# Autodesk Inventor assembly: docisk poprawne
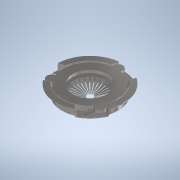
[picture p0: Inventor's stored thumbnail of the model, 180x180]
Saved by Autodesk Inventor 2022 (Build 260153000, 153)
## iProperties
Created: 2021-05-23
Part Number: docisk poprawne
Document SubType Name: Assembly
Designer: Matik
Author: Matik
## Documents named in this file (7)
- C:\Users\Mateu\Desktop\Modele\ClutchPressurePlate.iam
- C:\Users\Mateu\Desktop\Modele\ClutchPressurePlate_Casting.ipt
- C:\Users\Mateu\Desktop\Modele\ClutchPressurePlate_PlateSpring.ipt
- C:\Users\Mateu\Desktop\Modele\ClutchPressurePlate_TapeSpring.ipt
- C:\Users\Mateu\Desktop\Modele\ClutchPressurePlate_Cover.ipt
- C:\Users\Mateu\Desktop\Modele\ClutchPressurePlate_Rivet.ipt
- C:\Users\Mateu\Desktop\Modele\ClutchPressurePlate_RivetLong.ipt
## Components (12 placed, 6 different names)
1. ClutchPressurePlate_Casting:1 — Wstawiające:1, Wstawiające:2, Wstawiające:3, Wstawiające:4, Wstawiające:13
2. ClutchPressurePlate_PlateSpring:1 — Wstawiające:1
3. ClutchPressurePlate_TapeSpring:1 — Wstawiające:2, Wstawiające:6, Wstawiające:11
4. ClutchPressurePlate_TapeSpring:2 — Wstawiające:4, Wstawiające:7, Wstawiające:12
5. ClutchPressurePlate_TapeSpring:3 — Wstawiające:3, Wstawiające:5
6. ClutchPressurePlate_Cover:1 — Wstawiające:5, Wstawiające:6, Wstawiające:7, Wstawiające:8, Wstawiające:9, Wstawiające:10
7. ClutchPressurePlate_Rivet:1 — Wstawiające:8
8. ClutchPressurePlate_Rivet:2 — Wstawiające:9
9. ClutchPressurePlate_Rivet:3 — Wstawiające:10
10. ClutchPressurePlate_RivetLong:1 — Wstawiające:11
11. ClutchPressurePlate_RivetLong:2 — Wstawiające:13
12. ClutchPressurePlate_RivetLong:3 — Wstawiające:12
## Relationships (13: Insert 13)
- Wstawiające:1 [Insert]: ClutchPressurePlate_Casting:1 ↔ ClutchPressurePlate_PlateSpring:1
- Wstawiające:2 [Insert]: ClutchPressurePlate_Casting:1 ↔ ClutchPressurePlate_TapeSpring:1
- Wstawiające:3 [Insert]: ClutchPressurePlate_Casting:1 ↔ ClutchPressurePlate_TapeSpring:3
- Wstawiające:4 [Insert]: ClutchPressurePlate_Casting:1 ↔ ClutchPressurePlate_TapeSpring:2
- Wstawiające:5 [Insert]: ClutchPressurePlate_TapeSpring:3 ↔ ClutchPressurePlate_Cover:1
- Wstawiające:6 [Insert]: ClutchPressurePlate_TapeSpring:1 ↔ ClutchPressurePlate_Cover:1
- Wstawiające:7 [Insert]: ClutchPressurePlate_TapeSpring:2 ↔ ClutchPressurePlate_Cover:1
- Wstawiające:8 [Insert]: ClutchPressurePlate_Cover:1 ↔ ClutchPressurePlate_Rivet:1
- Wstawiające:9 [Insert]: ClutchPressurePlate_Cover:1 ↔ ClutchPressurePlate_Rivet:2
- Wstawiające:10 [Insert]: ClutchPressurePlate_Cover:1 ↔ ClutchPressurePlate_Rivet:3
- Wstawiające:11 [Insert]: ClutchPressurePlate_TapeSpring:1 ↔ ClutchPressurePlate_RivetLong:1
- Wstawiające:12 [Insert]: ClutchPressurePlate_TapeSpring:2 ↔ ClutchPressurePlate_RivetLong:3
- Wstawiające:13 [Insert]: ClutchPressurePlate_Casting:1 ↔ ClutchPressurePlate_RivetLong:2
